# Autodesk Inventor assembly: E000-Compresseur
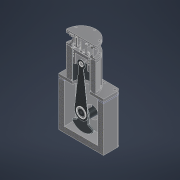
[picture p0: Inventor's stored thumbnail of the model, 180x180]
Saved by Autodesk Inventor 2021.3 (Build 253353000, 353)
## iProperties
Created: 2022-03-31
Part Number: E000-Compresseur
Document SubType Name: Assembly
Designer: remi
Author: remi
## Documents named in this file (11)
- C:\Users\remi\OneDrive\Documents\Cours\05-HEVS\S2fb\mechanic\CCo\project\Compressor\E000-Compresseur.iam
- C:\Users\remi\OneDrive\Documents\Cours\05-HEVS\S2fb\mechanic\CCo\project\Compressor\E001-Chambre.iam
- C:\Users\remi\OneDrive\Documents\Cours\05-HEVS\S2fb\mechanic\CCo\project\Compressor\E002-Piston.iam
- C:\Users\remi\OneDrive\Documents\Cours\05-HEVS\S2fb\mechanic\CCo\project\Compressor\E006-Carter.iam
- C:\Users\remi\OneDrive\Documents\Cours\05-HEVS\S2fb\mechanic\CCo\project\Compressor\P012-Bielle.ipt
- C:\Users\remi\OneDrive\Documents\Cours\05-HEVS\S2fb\mechanic\CCo\project\Compressor\Roulements\AIS2021\SKF_W 61701-2RS1.iam
- C:\Users\remi\OneDrive\Documents\Cours\05-HEVS\S2fb\mechanic\CCo\project\Compressor\Roulements\AIS2021\SKF_W 619_3-2Z.iam
- C:\Users\remi\OneDrive\Documents\Cours\05-HEVS\S2fb\mechanic\CCo\project\Compressor\E000-Compresseur\Design Accelerator\O-Ring1.iam
- C:\Users\remi\OneDrive\Documents\Cours\05-HEVS\S2fb\mechanic\CCo\project\Compressor\R2021\en-US\AS 1420\AS 1420 - 1973 - M4 x 12.ipt
- C:\Users\remi\OneDrive\Documents\Cours\05-HEVS\S2fb\mechanic\CCo\project\Compressor\R2021\en-US\AS 1420\AS 1420 - 1973 - M3 x 6.ipt
- C:\Users\remi\OneDrive\Documents\Cours\05-HEVS\S2fb\mechanic\CCo\project\Compressor\Compress Spring12.ipt
## Components (22 placed, 10 different names)
1. E001-Chambre:1 [sub-assembly] — Mate:1, Mate:17, Mate:18, Mate:19, Mate:20, Mate:21, Insert:24, Insert:25, Insert:26, Insert:27, Insert:28, Insert:29
2. E002-Piston:1 [sub-assembly] — Mate:1, Mate:15, Mate:16
3. E006-Carter:1 [sub-assembly] — Mate:12, Mate:14, Mate:17, Mate:18, Mate:19, Insert:16, Insert:17, Insert:18, Insert:19, Insert:20, Insert:21, Insert:22, Insert:23, Mate:22, Angle:1
4. P012-Bielle:1 — Mate:13, Mate:14, Flush:1, Mate:15, Insert:15
5. O-Ring:1 [sub-assembly] — Mate:20, Mate:21
6. Compress Spring1:1
7. AS 1420 - Metric M3 x 6:1 — Insert:24
8. AS 1420 - Metric M3 x 6:2 — Insert:25
9. AS 1420 - Metric M3 x 6:3 — Insert:26
10. AS 1420 - Metric M3 x 6:4 — Insert:27
11. AS 1420 - Metric M3 x 6:5 — Insert:28
12. AS 1420 - Metric M3 x 6:6 — Insert:29
13. AS 1420 - Metric M4 x 12:1 — Insert:16
14. AS 1420 - Metric M4 x 12:2 — Insert:17
15. AS 1420 - Metric M4 x 12:3 — Insert:18
16. AS 1420 - Metric M4 x 12:4 — Insert:19
17. AS 1420 - Metric M4 x 12:5 — Insert:20
18. AS 1420 - Metric M4 x 12:6 — Insert:21
19. AS 1420 - Metric M4 x 12:7 — Insert:22
20. AS 1420 - Metric M4 x 12:8 — Insert:23
21. SKF_W 619_3-2Z:1 [sub-assembly] — Mate:16, Insert:15
22. SKF_W 61701-2RS1:1 [sub-assembly] — Mate:12, Mate:13, Flush:1
## Relationships (29: Insert 15, Mate 12, Flush 1, Angle 1)
- Mate:1: E001-Chambre:1 ↔ E002-Piston:1
- Mate:12: E006-Carter:1 ↔ SKF_W 61701-2RS1:1
- Mate:13: P012-Bielle:1 ↔ SKF_W 61701-2RS1:1
- Mate:14: E006-Carter:1 ↔ P012-Bielle:1
- Flush:1: P012-Bielle:1 ↔ SKF_W 61701-2RS1:1
- Mate:15: E002-Piston:1 ↔ P012-Bielle:1
- Mate:16: E002-Piston:1 ↔ SKF_W 619_3-2Z:1
- Insert:15: P012-Bielle:1 ↔ SKF_W 619_3-2Z:1
- Mate:17: E001-Chambre:1 ↔ E006-Carter:1
- Mate:18: E001-Chambre:1 ↔ E006-Carter:1
- Mate:19: E001-Chambre:1 ↔ E006-Carter:1
- Mate:20: E001-Chambre:1 ↔ O-Ring:1
- Mate:21: E001-Chambre:1 ↔ O-Ring:1
- Insert:16: E006-Carter:1 ↔ AS 1420 - Metric M4 x 12:1
- Insert:17: E006-Carter:1 ↔ AS 1420 - Metric M4 x 12:2
- Insert:18: E006-Carter:1 ↔ AS 1420 - Metric M4 x 12:3
- Insert:19: E006-Carter:1 ↔ AS 1420 - Metric M4 x 12:4
- Insert:20: E006-Carter:1 ↔ AS 1420 - Metric M4 x 12:5
- Insert:21: E006-Carter:1 ↔ AS 1420 - Metric M4 x 12:6
- Insert:22: E006-Carter:1 ↔ AS 1420 - Metric M4 x 12:7
- Insert:23: E006-Carter:1 ↔ AS 1420 - Metric M4 x 12:8
- Mate:22: E006-Carter:1
- Angle:1 (0 deg): E006-Carter:1
- Insert:24: E001-Chambre:1 ↔ AS 1420 - Metric M3 x 6:1
- Insert:25: E001-Chambre:1 ↔ AS 1420 - Metric M3 x 6:2
- Insert:26: E001-Chambre:1 ↔ AS 1420 - Metric M3 x 6:3
- Insert:27: E001-Chambre:1 ↔ AS 1420 - Metric M3 x 6:4
- Insert:28: E001-Chambre:1 ↔ AS 1420 - Metric M3 x 6:5
- Insert:29: E001-Chambre:1 ↔ AS 1420 - Metric M3 x 6:6
